# Autodesk Inventor assembly: Assembly1
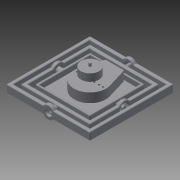
[picture p0: Inventor's stored thumbnail of the model, 180x180]
Saved by Autodesk Inventor 2015 (Build 190159000, 159)
## iProperties
Created: 2015-12-08
Part Number: Assembly1
Document SubType Name: Assembly
Designer: boztalay
Author: boztalay
## Documents named in this file (8)
- \\engin-labs.m.storage.umich.edu\boztalay\windat.V2\Documents\Inventor\HapticController\Assembly1.iam
- \\engin-labs.m.storage.umich.edu\boztalay\windat.V2\Documents\Inventor\HapticController\encoder.ipt
- \\engin-labs.m.storage.umich.edu\boztalay\windat.V2\Documents\Inventor\HapticController\motor.ipt
- \\engin-labs.m.storage.umich.edu\boztalay\windat.V2\Documents\Inventor\HapticController\knob.ipt
- \\engin-labs.m.storage.umich.edu\boztalay\windat.V2\Documents\Inventor\HapticController\shaft_adapter.ipt
- \\engin-labs.m.storage.umich.edu\boztalay\windat.V2\Documents\Inventor\HapticController\joystick_inner1.ipt
- \\engin-labs.m.storage.umich.edu\boztalay\windat.V2\Documents\Inventor\HapticController\joystick_outer.ipt
- \\engin-labs.m.storage.umich.edu\boztalay\windat.V2\Documents\Inventor\HapticController\joystick_mount.ipt
## Components (7 placed, 7 different names)
1. encoder:1 — Mate:4, Rigid:1
2. motor:1 — Insert:2, Mate:4
3. knob:1 — Mate:2, Mate:3, Flush:1
4. shaft_adapter:1 — Insert:2, Mate:2, Mate:3, Flush:1
5. joystick_inner1:1 — Rigid:1, Rotational:1
6. joystick_outer:1 — Rotational:1, Rotational:2
7. joystick_mount:1 — Rotational:2
## Relationships (8: Mate 3, RevoluteJoint 2, Insert 1, Flush 1, WeldJoint 1)
- Insert:2: motor:1 ↔ shaft_adapter:1
- Mate:2 (0.0889 mm): knob:1 ↔ shaft_adapter:1
- Mate:3 (0.0889 mm): knob:1 ↔ shaft_adapter:1
- Flush:1 (5.08 mm): knob:1 ↔ shaft_adapter:1
- Mate:4 (3.175 mm): encoder:1 ↔ motor:1
- Rigid:1 [WeldJoint]: encoder:1 ↔ joystick_inner1:1
- Rotational:1 [RevoluteJoint]: joystick_inner1:1 ↔ joystick_outer:1
- Rotational:2 [RevoluteJoint]: joystick_outer:1 ↔ joystick_mount:1
